# Autodesk Inventor assembly: Assembly Mount Assembly
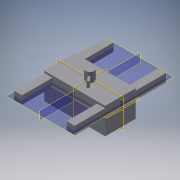
[picture p0: Inventor's stored thumbnail of the model, 180x180]
Saved by Autodesk Inventor 2019 (Build 230136000, 136)
## iProperties
Created: 2021-05-09
Part Number: Assembly Mount Assembly
Document SubType Name: Assembly
Designer: Eric
Author: Eric
## Documents named in this file (3)
- C:\Users\Eric\Documents\! - Uni\Year 4\MENG-Robot-Fab-Project\Models\For_Optimiser\Static Parts Assembly\Assembly Mount Assembly\Assembly Mount Assembly.iam
- C:\Users\Eric\Documents\! - Uni\Year 4\MENG-Robot-Fab-Project\Models\For_Optimiser\Static Parts Assembly\Assembly Mount Assembly\Assembly Mount Base.iam
- C:\Users\Eric\Documents\! - Uni\Year 4\MENG-Robot-Fab-Project\Models\For_Optimiser\Static Parts Assembly\Assembly Mount Assembly\Assembly Mount Rack.iam
## Components (2 placed, 2 different names)
1. Assembly Mount Base:2 [sub-assembly] — Mate:3, Mate:4, Mate:5
2. Assembly Mount Rack:2 [sub-assembly] — Mate:3, Mate:4, Mate:5
## Relationships (3: Mate 3)
- Mate:3: Assembly Mount Base:2 ↔ Assembly Mount Rack:2
- Mate:4: Assembly Mount Base:2 ↔ Assembly Mount Rack:2
- Mate:5 (11.5 mm): Assembly Mount Base:2 ↔ Assembly Mount Rack:2
